# Autodesk Inventor assembly: R-SO v11
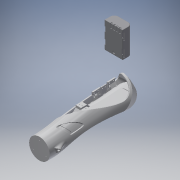
[picture p0: Inventor's stored thumbnail of the model, 180x180]
Saved by Autodesk Inventor 2018 (Build 220112000, 112)
## iProperties
Created: 2017-09-22
Part Number: R-SO v11
Material: 一般
Document SubType Name: Assembly
Designer: sktom
Author: sktom
## Documents named in this file (10)
- D:\cloudstrage\NextCloud\Cad_mechanical\HACKberry_SizeM\3Dmodel\R\M-R-SO\M-R-SO.iam
- D:\cloudstrage\NextCloud\Cad_mechanical\HACKberry_SizeM\3Dmodel\R\M-R-SO\M-R-SO-02.ipt
- D:\cloudstrage\NextCloud\Cad_mechanical\HACKberry_SizeM\3Dmodel\R\M-R-SO\M-R-SO-01.ipt
- D:\cloudstrage\NextCloud\Cad_mechanical\HACKberry_SizeM\3Dmodel\R\M-R-SO\M-R-SO-05.ipt
- D:\cloudstrage\NextCloud\Cad_mechanical\HACKberry_SizeM\3Dmodel\R\M-R-SO\M-R-SO-06.ipt
- D:\cloudstrage\NextCloud\Cad_mechanical\HACKberry_SizeM\3Dmodel\R\M-R-SO\M-R-SO-07.ipt
- D:\cloudstrage\NextCloud\Cad_mechanical\HACKberry_SizeM\3Dmodel\R\M-R-SO\M-R-SO-08.ipt
- D:\cloudstrage\NextCloud\Cad_mechanical\HACKberry_SizeM\3Dmodel\R\M-R-SO\M-R-SO-09.ipt
- D:\cloudstrage\NextCloud\Cad_mechanical\HACKberry_SizeM\3Dmodel\R\M-R-SO\M-R-SO-10.ipt
- D:\cloudstrage\NextCloud\Cad_mechanical\HACKberry_SizeM\3Dmodel\R\M-R-SO\DMW-BLF19.ipt
## Components (9 placed, 9 different names)
1. R-SO-02 v2:1 — リジッド:2
2. R-SO-01 v2:1 — リジッド:2
3. R-SO-05 v2:1
4. R-SO-06 v2:1
5. R-SO-07 v2:1
6. R-SO-08 v2:1
7. R-SO-09 v2:1
8. R-SO-10 v2:1
9. DMW-BLF19:1
## Relationships (1: WeldJoint 1)
- リジッド:2 [WeldJoint] (-0.14 mm): R-SO-02 v2:1 ↔ R-SO-01 v2:1
